# Autodesk Inventor assembly: 14-3
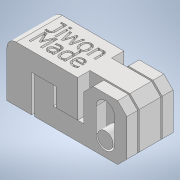
[picture p0: Inventor's stored thumbnail of the model, 180x180]
Saved by Autodesk Inventor 2022 (Build 260153000, 153)
## iProperties
Created: 2021-09-12
Part Number: 14-3
Document SubType Name: Assembly
Designer: 서울공업고등학교
Author: 서울공업고등학교
## Documents named in this file (3)
- C:\Users\서울공업고등학교\Documents\_9_12\모의고사14\14-3.iam
- C:\Users\서울공업고등학교\Documents\_9_12\모의고사14\14-1.ipt
- C:\Users\서울공업고등학교\Documents\_9_12\모의고사14\14-2.ipt
## Components (2 placed, 2 different names)
1. 14-1:1 — 플러쉬:1, 메이트:1
2. 14-2:1 — 플러쉬:1, 메이트:1
## Relationships (2: Flush 1, Mate 1)
- 플러쉬:1 [Flush]: 14-1:1 ↔ 14-2:1
- 메이트:1 [Mate]: 14-1:1 ↔ 14-2:1
